# Autodesk Inventor assembly: Ensamble Sistema Bandeja Almacenamiento
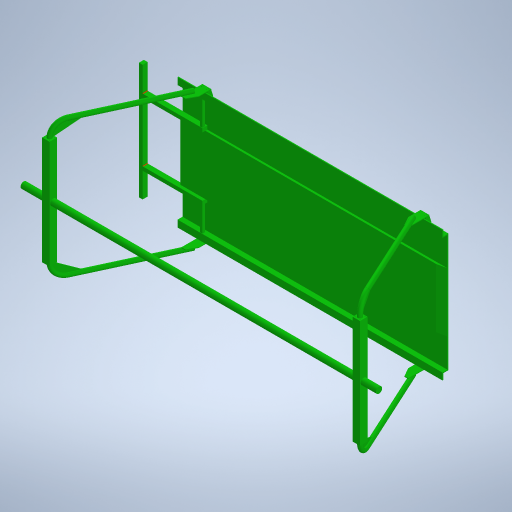
[picture p0: Inventor's stored thumbnail of the model, 512x512]
Saved by Autodesk Inventor 2024.3 (Build 283343000, 343)
## iProperties
Created: 2025-05-04
Part Number: Ensamble Sistema Bandeja Almacenamiento
Document SubType Name: Assembly
Designer: Gary
Author: Gary
## Documents named in this file (7)
- C:\Users\Windows11\Desktop\motor de trasmision de potencia\Sistema de Bandeja de Almacenamiento\Ensamble Sistema Bandeja Almacenamiento.iam
- C:\Users\Windows11\Desktop\motor de trasmision de potencia\Sistema de Bandeja de Almacenamiento\Bandeja Soporte Automovil.ipt
- C:\Users\Windows11\Desktop\motor de trasmision de potencia\Sistema de Bandeja de Almacenamiento\Soporte Lateral.ipt
- C:\Users\Windows11\Desktop\motor de trasmision de potencia\Sistema de Bandeja de Almacenamiento\Soporte Lateral_MIR.ipt
- C:\Users\Windows11\Desktop\motor de trasmision de potencia\Sistema de Bandeja de Almacenamiento\Soporte Lateral_MIR1.ipt
- C:\Users\Windows11\Desktop\motor de trasmision de potencia\Sistema de Bandeja de Almacenamiento\Soporte Lateral_MIR_MIR.ipt
- C:\Users\Windows11\Desktop\motor de trasmision de potencia\Sistema de Bandeja de Almacenamiento\Soporte Superior bandeja.ipt
## Components (6 placed, 6 different names)
1. Bandeja Soporte Automovil:1 — Flush:1, Mate:1, Flush:2, Mate:2, Flush:3, Flush:4, Mate:3, Insert:1, Mate:4, Mate:5, Insert:2, Insert:3
2. Soporte Lateral:1 — Flush:1, Mate:1, Flush:2, Mate:2
3. Soporte Lateral_MIR:1 — Mate:5, Insert:2, Mate:6
4. Soporte Lateral_MIR1:1 — Flush:3, Mate:3, Insert:1
5. Soporte Lateral_MIR_MIR:1 — Flush:4, Mate:4, Insert:3, Flush:5, Flush:6, Mate:7, Flush:7, Flush:8
6. Soporte Superior bandeja:1 — Mate:6, Flush:5, Flush:6, Mate:7, Flush:7, Flush:8
## Relationships (18: Flush 8, Mate 7, Insert 3)
- Flush:1: Bandeja Soporte Automovil:1 ↔ Soporte Lateral:1
- Mate:1: Bandeja Soporte Automovil:1 ↔ Soporte Lateral:1
- Flush:2: Bandeja Soporte Automovil:1 ↔ Soporte Lateral:1
- Mate:2: Bandeja Soporte Automovil:1 ↔ Soporte Lateral:1
- Flush:3: Bandeja Soporte Automovil:1 ↔ Soporte Lateral_MIR1:1
- Flush:4: Bandeja Soporte Automovil:1 ↔ Soporte Lateral_MIR_MIR:1
- Mate:3: Bandeja Soporte Automovil:1 ↔ Soporte Lateral_MIR1:1
- Insert:1: Bandeja Soporte Automovil:1 ↔ Soporte Lateral_MIR1:1
- Mate:4: Bandeja Soporte Automovil:1 ↔ Soporte Lateral_MIR_MIR:1
- Mate:5: Bandeja Soporte Automovil:1 ↔ Soporte Lateral_MIR:1
- Insert:2: Bandeja Soporte Automovil:1 ↔ Soporte Lateral_MIR:1
- Insert:3: Bandeja Soporte Automovil:1 ↔ Soporte Lateral_MIR_MIR:1
- Mate:6: Soporte Lateral_MIR:1 ↔ Soporte Superior bandeja:1
- Flush:5: Soporte Lateral_MIR_MIR:1 ↔ Soporte Superior bandeja:1
- Flush:6: Soporte Lateral_MIR_MIR:1 ↔ Soporte Superior bandeja:1
- Mate:7: Soporte Lateral_MIR_MIR:1 ↔ Soporte Superior bandeja:1
- Flush:7: Soporte Lateral_MIR_MIR:1 ↔ Soporte Superior bandeja:1
- Flush:8: Soporte Lateral_MIR_MIR:1 ↔ Soporte Superior bandeja:1
